# Autodesk Inventor assembly: gear_MIR
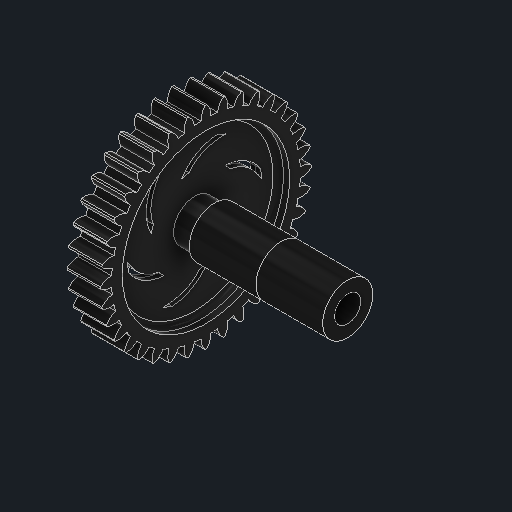
[picture p0: Inventor's stored thumbnail of the model, 512x512]
Saved by Autodesk Inventor 2024 (Build 280153000, 153)
## iProperties
Created: 2023-10-18
Part Number: gear_MIR
Document SubType Name: Assembly
Designer: Averey Ku
Author: Averey Ku
## Documents named in this file (4)
- D:\vex_robotics\hardware\cad\goated_v0.1\chassis\mirrored_parts\gear_MIR.iam
- D:\vex_robotics\hardware\cad\VEX-CAD-Inventor-1.41\Motion\Spacers\Spacer Nylon .375 OD\NSpacer .375 OD x .500.ipt
- D:\vex_robotics\hardware\cad\VEX-CAD-Inventor-1.41\Motion\Spacers\Spacer Nylon .375 OD.ipt
- D:\vex_robotics\hardware\cad\goated_v0.1\chassis\mirrored_parts\LS 36T Gear_MIR.ipt
## Components (3 placed, 2 different names)
1. NSpacer .375 OD x .500:1 — Insert:1
2. NSpacer .375 OD x .500:2 — Insert:1, Insert:2
3. LS 36T Gear_MIR:1 — Insert:2
## Relationships (2: Insert 2)
- Insert:1: NSpacer .375 OD x .500:1 ↔ NSpacer .375 OD x .500:2
- Insert:2: NSpacer .375 OD x .500:2 ↔ LS 36T Gear_MIR:1
